# Autodesk Inventor assembly: EE_base_assembly
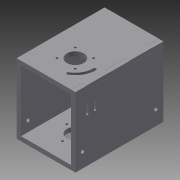
[picture p0: Inventor's stored thumbnail of the model, 180x180]
Saved by Autodesk Inventor 2015 (Build 190159000, 159)
## iProperties
Created: 2017-03-04
Part Number: EE_base_assembly
Document SubType Name: Assembly
Designer: Guy
Author: Guy
## Documents named in this file (5)
- C:\Users\Ernest\Documents\Capstone-Project\doc\CAD\LowLevel_Rev3\EE_base\EE_base_assembly.iam
- C:\Users\Ernest\Documents\Capstone-Project\doc\CAD\LowLevel_Rev3\EE_base\bottom.ipt
- C:\Users\Ernest\Documents\Capstone-Project\doc\CAD\LowLevel_Rev3\EE_base\top.ipt
- C:\Users\Ernest\Documents\Capstone-Project\doc\CAD\LowLevel_Rev3\EE_base\SideLeft.ipt
- C:\Users\Ernest\Documents\Capstone-Project\doc\CAD\LowLevel_Rev3\EE_base\SideRight.ipt
## Components (4 placed, 4 different names)
1. bottom:1 — Mate:1, Flush:3, Mate:4
2. top:1 — Mate:2, Flush:4, Mate:3, Mate:5
3. SideLeft:1 — Flush:1, Flush:2, Mate:1, Flush:3, Mate:2, Flush:4, Mate:3, Mate:4
4. SideRight:1 — Flush:1, Flush:2, Mate:5
## Relationships (9: Mate 5, Flush 4)
- Flush:1: SideLeft:1 ↔ SideRight:1
- Flush:2: SideLeft:1 ↔ SideRight:1
- Mate:1: bottom:1 ↔ SideLeft:1
- Flush:3: bottom:1 ↔ SideLeft:1
- Mate:2: top:1 ↔ SideLeft:1
- Flush:4: top:1 ↔ SideLeft:1
- Mate:3: top:1 ↔ SideLeft:1
- Mate:4: bottom:1 ↔ SideLeft:1
- Mate:5: top:1 ↔ SideRight:1
